# Autodesk Inventor assembly: RCPlaneAssembly1
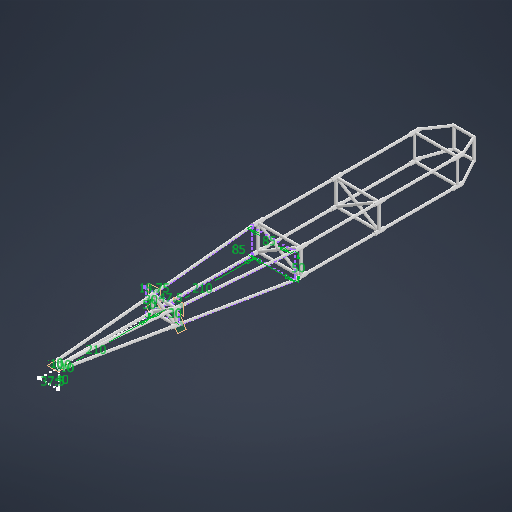
[picture p0: Inventor's stored thumbnail of the model, 512x512]
Saved by Autodesk Inventor 2026.1 (Build 301233000, 233)
## iProperties
Created: 2026-03-11
Part Number: RCPlaneAssembly1
Document SubType Name: Assembly
Designer: morri
Author: morri
## Documents named in this file (5)
- C:\Users\morri\Documents\ENGR 2999 (Capstone)\RCPlaneAssembly1.iam
- C:\Users\morri\Documents\ENGR 2999 (Capstone)\RCPlaneSkeletonTailFront.ipt
- C:\Users\morri\Documents\ENGR 2999 (Capstone)\RCPlaneSkeletonMiddleFront2.ipt
- C:\Users\morri\Documents\ENGR 2999 (Capstone)\RCPlaneTailRear2.ipt
- C:\Users\morri\Documents\ENGR 2999 (Capstone)\RCPlaneSkeletonFront2.ipt
## Components (5 placed, 4 different names)
1. RCPlaneSkeletonTailFront:1 — Insert:5, Insert:6
2. RCPlaneSkeletonMiddleFront2:1 — Insert:4, Insert:7
3. RCPlaneSkeletonMiddleFront2:2 — Insert:4, Insert:5
4. RCPlaneTailRear2:1 — Insert:6
5. RCPlaneSkeletonFront2:1 — Insert:7
## Relationships (4: Insert 4)
- Insert:4: RCPlaneSkeletonMiddleFront2:1 ↔ RCPlaneSkeletonMiddleFront2:2
- Insert:5: RCPlaneSkeletonTailFront:1 ↔ RCPlaneSkeletonMiddleFront2:2
- Insert:6: RCPlaneSkeletonTailFront:1 ↔ RCPlaneTailRear2:1
- Insert:7: RCPlaneSkeletonMiddleFront2:1 ↔ RCPlaneSkeletonFront2:1
